# Autodesk Inventor assembly: motor-mount
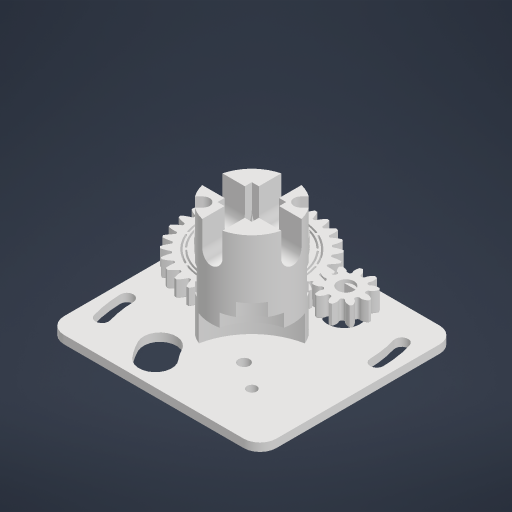
[picture p0: Inventor's stored thumbnail of the model, 512x512]
Saved by Autodesk Inventor 2024 (Build 280153000, 153)
## iProperties
Created: 2024-05-16
Part Number: motor-mount
Document SubType Name: Assembly
Designer: loren
elephant_prevention_radius: 0,300 mm
Author: loren
## Documents named in this file (8)
- C:\Users\lokies\Nextcloud\projects\motorized-mounts\mechanical\cheap-geared\cheap-geared.iam
- C:\Users\lokies\Nextcloud\projects\motorized-mounts\mechanical\cheap-geared\mount-plate.ipt
- C:\Users\lokies\Nextcloud\projects\motorized-mounts\mechanical\cheap-geared\gear.ipt
- C:\Users\lokies\Nextcloud\projects\motorized-mounts\mechanical\cheap-geared\screw-grip.ipt
- C:\Users\lokies\Nextcloud\projects\motorized-mounts\mechanical\cheap-geared\mount-stem.ipt
- C:\Users\lokies\Nextcloud\projects\motorized-mounts\mechanical\cheap-geared\pinion.ipt
- C:\Users\lokies\Nextcloud\projects\motorized-mounts\mechanical\cheap-geared\washer.ipt
- C:\Users\lokies\Nextcloud\projects\motorized-mounts\mechanical\cheap-geared\params.xlsx
## Components (6 placed, 6 different names)
1. mount-plate:1 — Mate:1, Mate:2, Mate:4, Mate:5, Flush:3, Mate:6, Mate:8
2. gear:1 — Mate:1, Mate:2, Mate:3, Flush:1, Flush:2, Mate:7, Flush:4, Flush:5, Mate:9
3. screw-grip:1 — Mate:3, Flush:1, Flush:2
4. mount-stem:1 — Mate:4, Mate:5, Flush:3
5. pinion:1 — Mate:6, Mate:7, Mate:8
6. washer:1 — Flush:4, Flush:5, Mate:9
## Relationships (14: Mate 9, Flush 5)
- Mate:1: mount-plate:1 ↔ gear:1
- Mate:2 (1 mm): mount-plate:1 ↔ gear:1
- Mate:3: gear:1 ↔ screw-grip:1
- Flush:1: gear:1 ↔ screw-grip:1
- Flush:2: gear:1 ↔ screw-grip:1
- Mate:4: mount-plate:1 ↔ mount-stem:1
- Mate:5: mount-plate:1 ↔ mount-stem:1
- Flush:3: mount-plate:1 ↔ mount-stem:1
- Mate:6 (0.5 mm): mount-plate:1 ↔ pinion:1
- Mate:7 (25 mm): gear:1 ↔ pinion:1
- Mate:8 (19.2419 mm): mount-plate:1 ↔ pinion:1
- Flush:4: gear:1 ↔ washer:1
- Flush:5: gear:1 ↔ washer:1
- Mate:9: gear:1 ↔ washer:1
## Named parameters: thumbscrew_dia = 15.8 mm, helix_length = 3.5 mm, helix_width = 2 mm, helix_fillet = 0.3 mm, helix_teeth = 8, helix_inner_dia = 19 mm, helix_outer_dia = 23 mm, elephant_prevention_radius = 0.3 mm, gear_center_distance = 25 mm, stepper_screw_dist = 35 mm, stepper_axis_offset = 8 mm, stepper_axis_clearance = 10 mm, mount_screw_ortho_dist = 31 mm, stepper_dia = 28 mm, sheet_thick = 2.5 mm, helix_winding_factor = 1.2
